# Autodesk Inventor assembly: 1725850 EAGF-V2-KF-100-100---(0)
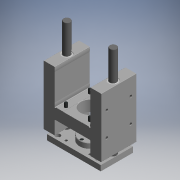
[picture p0: Inventor's stored thumbnail of the model, 180x180]
Saved by Autodesk Inventor 2017.3 (Build 213256000, 256)
## iProperties
Category: PARTsolutions
Company: FESTO
Part Number: 1725850 EAGF-V2-KF-100-100---(0)
Catalog Web Link: www.cadenas.de
Description: EAGF-guide unit
Vendor: FESTO
Document SubType Name: Assembly
Designer: partserver
Manufacturer: FESTO
Mass: 14023 g
Surface Area: 4822.3 cm^2
Volume: 3416.6 cm^3
Density: 4.10438 g/cm^3
Title: 1725850 EAGF-V2-KF-100-100
Author: Cadenas PARTsolutions
Comments: guide unit
PSOL_IDENT_0: {ATYP=ASSISTANT},{DATA=script=$CADENAS_DATA/23d-libs/festo/webfesto.vbb&M_FAMILY=EAGF&M_GROUP=01&M_P
PSOL_IDENT_1: ARTNO=1725850&IDCODE1=EAGF-V2-KF-100-100&IDCODE2=&customer_number_cns=&MATES=1&LOD=HI&LOCKERP=0&SING
PSOL_IDENT_2: LEPART=1}
NB: 1725850 EAGF-V2-KF-100-100---(0)
NN: EAGF
NT: guide unit
NBSYN: $TNR. $TYP.---($HUBST.)
LINA: 1725850 EAGF-V2-KF-100-100
CATALOG: Festo
TNR: 1725850
TYP: EAGF-V2-KF-100-100
HUBST: 0
L1: 362.8
L2: 126.6
L3: 220
L4: 40
L5: 128
L6: 20
L7: 24.5
L8: 89
L9: 0
L10: 15
L11: 39
H1: 213
H2: 200
H3: 89
H4: 150
H5: 131
H6: 172
H7: 150
B1: 130
B2: 120
B3: 89
B4: 89
B5: 89
D1: 87
D2: 25
D3: 18
D4: 11
D5: 70
KK: M20x1.5
G1: M18
G2: M10
G3: M10
T1: 20
T2: 11
SW: 27
CNSMASSEXACT: 14.023
SUPPLIER: FESTO
ARTICLENO: 1725850 EAGF-V2-KF-100-100---(0)
BOMINFO: 1725850 EAGF-V2-KF-100-100
CREATOR: CADENAS GmbH
## Documents named in this file (12)
- e:\temp\worker_18\temp\exporttempdir_1120_80_rasIC\format_0\1725850 EAGF-V2-KF-100-100---(0).iam
- e:\temp\worker_18\temp\exporttempdir_1120_80_rasIC\format_0\2608532 EAGF-V2-KF-100---(F).ipt
- e:\temp\worker_18\temp\exporttempdir_1120_80_rasIC\format_0\247465 FEN-80-SD---(SD).ipt
- e:\temp\worker_18\temp\exporttempdir_1120_80_rasIC\format_0\242770 EAGF 25x35x40---(B).ipt
- e:\temp\worker_18\temp\exporttempdir_1120_80_rasIC\format_0\1558863 EAGF-V2-KF-100---(J).ipt
- e:\temp\worker_18\temp\exporttempdir_1120_80_rasIC\format_0\1559396 EAGF-V2-KF-100---(R).ipt
- e:\temp\worker_18\temp\exporttempdir_1120_80_rasIC\format_0\1559400 EAGF-V2-KF-80_100---(GS).ipt
- e:\temp\worker_18\temp\exporttempdir_1120_80_rasIC\format_0\DIN-913 - M18x20.ipt
- e:\temp\worker_18\temp\exporttempdir_1120_80_rasIC\format_0\2608532 EAGF-100-100-KF---(FST).ipt
- e:\temp\worker_18\temp\exporttempdir_1120_80_rasIC\format_0\DIN-912 - M12x25(F).ipt
- e:\temp\worker_18\temp\exporttempdir_1120_80_rasIC\format_0\DIN-6912 - M12x25(F).ipt
- e:\temp\worker_18\temp\exporttempdir_1120_80_rasIC\format_0\DIN-912 - M10x50(F).ipt
## Components (25 placed, 11 different names)
1. 2608532 EAGF-V2-KF-100---(F):1 — ABSTREIF_V_1_XY@1 <-> ANBAU_XY@2, ABSTREIF_V_1_Z@1 <-> ANBAU_Z@2, ABSTREIF_V_1_YZ@1 <-> ANBAU_YZ@2, ABSTREIF_V_2_XY@1 <-> ANBAU_XY@3, ABSTREIF_V_2_Z@1 <-> ANBAU_Z@3, ABSTREIF_V_2_YZ@1 <-> ANBAU_YZ@3, BUSH_V_1_XY@1 <-> ANBAU_XY@4, BUSH_V_1_Z@1 <-> ANBAU_Z@4, BUSH_V_1_YZ@1 <-> ANBAU_YZ@4, BUSH_V_2_XY@1 <-> ANBAU_XY@5, BUSH_V_2_Z@1 <-> ANBAU_Z@5, BUSH_V_2_YZ@1 <-> ANBAU_YZ@5, ABSTREIF_H_1_XY@1 <-> ANBAU_XY@6, ABSTREIF_H_1_Z@1 <-> ANBAU_Z@6, ABSTREIF_H_1_YZ@1 <-> ANBAU_YZ@6, ABSTREIF_H_2_XY@1 <-> ANBAU_XY@7, ABSTREIF_H_2_Z@1 <-> ANBAU_Z@7, ABSTREIF_H_2_YZ@1 <-> ANBAU_YZ@7, BUSH_H_1_XY@1 <-> ANBAU_XY@8, BUSH_H_1_Z@1 <-> ANBAU_Z@8, BUSH_H_1_YZ@1 <-> ANBAU_YZ@8, BUSH_H_2_XY@1 <-> ANBAU_XY@9, BUSH_H_2_Z@1 <-> ANBAU_Z@9, BUSH_H_2_YZ@1 <-> ANBAU_YZ@9, JOCH_Z@1 <-> ANBAU_Z@10, JOCH_YZ@1 <-> ANBAU_YZ@10, DIN912_1_Z@1 <-> ANBAU_Z@22, DIN912_2_Z@1 <-> ANBAU_Z@23, DIN912_3_Z@1 <-> ANBAU_Z@24, DIN912_4_Z@1 <-> ANBAU_Z@25
2. 247465 FEN-80-SD---(SD):1 — ABSTREIF_V_1_XY@1 <-> ANBAU_XY@2, ABSTREIF_V_1_Z@1 <-> ANBAU_Z@2, ABSTREIF_V_1_YZ@1 <-> ANBAU_YZ@2
3. 247465 FEN-80-SD---(SD):2 — ABSTREIF_V_2_XY@1 <-> ANBAU_XY@3, ABSTREIF_V_2_Z@1 <-> ANBAU_Z@3, ABSTREIF_V_2_YZ@1 <-> ANBAU_YZ@3
4. 242770 EAGF 25x35x40---(B):1 — BUSH_V_1_XY@1 <-> ANBAU_XY@4, BUSH_V_1_Z@1 <-> ANBAU_Z@4, BUSH_V_1_YZ@1 <-> ANBAU_YZ@4
5. 242770 EAGF 25x35x40---(B):2 — BUSH_V_2_XY@1 <-> ANBAU_XY@5, BUSH_V_2_Z@1 <-> ANBAU_Z@5, BUSH_V_2_YZ@1 <-> ANBAU_YZ@5
6. 247465 FEN-80-SD---(SD):3 — ABSTREIF_H_1_XY@1 <-> ANBAU_XY@6, ABSTREIF_H_1_Z@1 <-> ANBAU_Z@6, ABSTREIF_H_1_YZ@1 <-> ANBAU_YZ@6
7. 247465 FEN-80-SD---(SD):4 — ABSTREIF_H_2_XY@1 <-> ANBAU_XY@7, ABSTREIF_H_2_Z@1 <-> ANBAU_Z@7, ABSTREIF_H_2_YZ@1 <-> ANBAU_YZ@7
8. 242770 EAGF 25x35x40---(B):3 — BUSH_H_1_XY@1 <-> ANBAU_XY@8, BUSH_H_1_Z@1 <-> ANBAU_Z@8, BUSH_H_1_YZ@1 <-> ANBAU_YZ@8
9. 242770 EAGF 25x35x40---(B):4 — BUSH_H_2_XY@1 <-> ANBAU_XY@9, BUSH_H_2_Z@1 <-> ANBAU_Z@9, BUSH_H_2_YZ@1 <-> ANBAU_YZ@9
10. 1558863 EAGF-V2-KF-100---(J):1 — JOCH_Z@1 <-> ANBAU_Z@10, JOCH_YZ@1 <-> ANBAU_YZ@10, RING_XY@10 <-> ANBAU_XY@11, RING_Z@10 <-> ANBAU_Z@11, RING_YZ@10 <-> ANBAU_YZ@11, STANGE_XY@10 <-> ANBAU_XY@14, STANGE_Z@10 <-> ANBAU_Z@14, STANGE_2_XY@10 <-> ANBAU_XY@15, STANGE_2_Z@10 <-> ANBAU_Z@15, SCREW_1_XY@10 <-> ANBAU_XY@16, SCREW_1_Z@10 <-> ANBAU_Z@16, SCREW_1_YZ@10 <-> ANBAU_YZ@16, SCREW_2_XY@10 <-> ANBAU_XY@17, SCREW_2_Z@10 <-> ANBAU_Z@17, SCREW_2_YZ@10 <-> ANBAU_YZ@17, SCREW_3_XY@10 <-> ANBAU_XY@18, SCREW_3_Z@10 <-> ANBAU_Z@18, SCREW_3_YZ@10 <-> ANBAU_YZ@18, SCREW_4_XY@10 <-> ANBAU_XY@19, SCREW_4_Z@10 <-> ANBAU_Z@19, SCREW_4_YZ@10 <-> ANBAU_YZ@19, DIN6912_1_XY@10 <-> MONTAGE_XY@20, DIN6912_1_Z@10 <-> MONTAGE_Z@20, DIN6912_2_XY@10 <-> MONTAGE_XY@21, DIN6912_2_Z@10 <-> MONTAGE_Z@21
11. 1559396 EAGF-V2-KF-100---(R):1 — RING_XY@10 <-> ANBAU_XY@11, RING_Z@10 <-> ANBAU_Z@11, RING_YZ@10 <-> ANBAU_YZ@11, EP_IP_XY@11 <-> ANBAU_XY@12, EP_IP_Z@11 <-> ANBAU_Z@12, EP_IP_YZ@11 <-> ANBAU_YZ@12
12. 1559400 EAGF-V2-KF-80_100---(GS):1 — EP_IP_XY@11 <-> ANBAU_XY@12, EP_IP_Z@11 <-> ANBAU_Z@12, EP_IP_YZ@11 <-> ANBAU_YZ@12, EP_IP_Z@12 <-> IP2_Z@13
13. DIN-913 - M18x20:1 — EP_IP_Z@12 <-> IP2_Z@13
14. 2608532 EAGF-100-100-KF---(FST):1 — STANGE_XY@10 <-> ANBAU_XY@14, STANGE_Z@10 <-> ANBAU_Z@14
15. 2608532 EAGF-100-100-KF---(FST):2 — STANGE_2_XY@10 <-> ANBAU_XY@15, STANGE_2_Z@10 <-> ANBAU_Z@15
16. DIN-912 - M12x25(F):1 — SCREW_1_XY@10 <-> ANBAU_XY@16, SCREW_1_Z@10 <-> ANBAU_Z@16, SCREW_1_YZ@10 <-> ANBAU_YZ@16
17. DIN-912 - M12x25(F):2 — SCREW_2_XY@10 <-> ANBAU_XY@17, SCREW_2_Z@10 <-> ANBAU_Z@17, SCREW_2_YZ@10 <-> ANBAU_YZ@17
18. DIN-912 - M12x25(F):3 — SCREW_3_XY@10 <-> ANBAU_XY@18, SCREW_3_Z@10 <-> ANBAU_Z@18, SCREW_3_YZ@10 <-> ANBAU_YZ@18
19. DIN-912 - M12x25(F):4 — SCREW_4_XY@10 <-> ANBAU_XY@19, SCREW_4_Z@10 <-> ANBAU_Z@19, SCREW_4_YZ@10 <-> ANBAU_YZ@19
20. DIN-6912 - M12x25(F):1 — DIN6912_1_XY@10 <-> MONTAGE_XY@20, DIN6912_1_Z@10 <-> MONTAGE_Z@20
21. DIN-6912 - M12x25(F):2 — DIN6912_2_XY@10 <-> MONTAGE_XY@21, DIN6912_2_Z@10 <-> MONTAGE_Z@21
22. DIN-912 - M10x50(F):1 — DIN912_1_Z@1 <-> ANBAU_Z@22
23. DIN-912 - M10x50(F):2 — DIN912_2_Z@1 <-> ANBAU_Z@23
24. DIN-912 - M10x50(F):3 — DIN912_3_Z@1 <-> ANBAU_Z@24
25. DIN-912 - M10x50(F):4 — DIN912_4_Z@1 <-> ANBAU_Z@25
## Relationships (57: Mate 36, Angle 15, Flush 6)
- ABSTREIF_V_1_XY@1 <-> ANBAU_XY@2 [Mate]: 2608532 EAGF-V2-KF-100---(F):1 ↔ 247465 FEN-80-SD---(SD):1
- ABSTREIF_V_1_Z@1 <-> ANBAU_Z@2 [Mate]: 2608532 EAGF-V2-KF-100---(F):1 ↔ 247465 FEN-80-SD---(SD):1
- ABSTREIF_V_1_YZ@1 <-> ANBAU_YZ@2 [Angle] (0 deg): 2608532 EAGF-V2-KF-100---(F):1 ↔ 247465 FEN-80-SD---(SD):1
- ABSTREIF_V_2_XY@1 <-> ANBAU_XY@3 [Mate]: 2608532 EAGF-V2-KF-100---(F):1 ↔ 247465 FEN-80-SD---(SD):2
- ABSTREIF_V_2_Z@1 <-> ANBAU_Z@3 [Mate]: 2608532 EAGF-V2-KF-100---(F):1 ↔ 247465 FEN-80-SD---(SD):2
- ABSTREIF_V_2_YZ@1 <-> ANBAU_YZ@3 [Angle] (0 deg): 2608532 EAGF-V2-KF-100---(F):1 ↔ 247465 FEN-80-SD---(SD):2
- BUSH_V_1_XY@1 <-> ANBAU_XY@4 [Mate]: 2608532 EAGF-V2-KF-100---(F):1 ↔ 242770 EAGF 25x35x40---(B):1
- BUSH_V_1_Z@1 <-> ANBAU_Z@4 [Mate]: 2608532 EAGF-V2-KF-100---(F):1 ↔ 242770 EAGF 25x35x40---(B):1
- BUSH_V_1_YZ@1 <-> ANBAU_YZ@4 [Angle] (0 deg): 2608532 EAGF-V2-KF-100---(F):1 ↔ 242770 EAGF 25x35x40---(B):1
- BUSH_V_2_XY@1 <-> ANBAU_XY@5 [Mate]: 2608532 EAGF-V2-KF-100---(F):1 ↔ 242770 EAGF 25x35x40---(B):2
- BUSH_V_2_Z@1 <-> ANBAU_Z@5 [Mate]: 2608532 EAGF-V2-KF-100---(F):1 ↔ 242770 EAGF 25x35x40---(B):2
- BUSH_V_2_YZ@1 <-> ANBAU_YZ@5 [Angle] (0 deg): 2608532 EAGF-V2-KF-100---(F):1 ↔ 242770 EAGF 25x35x40---(B):2
- ABSTREIF_H_1_XY@1 <-> ANBAU_XY@6 [Mate]: 2608532 EAGF-V2-KF-100---(F):1 ↔ 247465 FEN-80-SD---(SD):3
- ABSTREIF_H_1_Z@1 <-> ANBAU_Z@6 [Mate]: 2608532 EAGF-V2-KF-100---(F):1 ↔ 247465 FEN-80-SD---(SD):3
- ABSTREIF_H_1_YZ@1 <-> ANBAU_YZ@6 [Angle] (0 deg): 2608532 EAGF-V2-KF-100---(F):1 ↔ 247465 FEN-80-SD---(SD):3
- ABSTREIF_H_2_XY@1 <-> ANBAU_XY@7 [Mate]: 2608532 EAGF-V2-KF-100---(F):1 ↔ 247465 FEN-80-SD---(SD):4
- ABSTREIF_H_2_Z@1 <-> ANBAU_Z@7 [Mate]: 2608532 EAGF-V2-KF-100---(F):1 ↔ 247465 FEN-80-SD---(SD):4
- ABSTREIF_H_2_YZ@1 <-> ANBAU_YZ@7 [Angle] (0 deg): 2608532 EAGF-V2-KF-100---(F):1 ↔ 247465 FEN-80-SD---(SD):4
- BUSH_H_1_XY@1 <-> ANBAU_XY@8 [Mate]: 2608532 EAGF-V2-KF-100---(F):1 ↔ 242770 EAGF 25x35x40---(B):3
- BUSH_H_1_Z@1 <-> ANBAU_Z@8 [Mate]: 2608532 EAGF-V2-KF-100---(F):1 ↔ 242770 EAGF 25x35x40---(B):3
- BUSH_H_1_YZ@1 <-> ANBAU_YZ@8 [Angle] (0 deg): 2608532 EAGF-V2-KF-100---(F):1 ↔ 242770 EAGF 25x35x40---(B):3
- BUSH_H_2_XY@1 <-> ANBAU_XY@9 [Mate]: 2608532 EAGF-V2-KF-100---(F):1 ↔ 242770 EAGF 25x35x40---(B):4
- BUSH_H_2_Z@1 <-> ANBAU_Z@9 [Mate]: 2608532 EAGF-V2-KF-100---(F):1 ↔ 242770 EAGF 25x35x40---(B):4
- BUSH_H_2_YZ@1 <-> ANBAU_YZ@9 [Angle] (0 deg): 2608532 EAGF-V2-KF-100---(F):1 ↔ 242770 EAGF 25x35x40---(B):4
- JOCH_Z@1 <-> ANBAU_Z@10 [Mate]: 2608532 EAGF-V2-KF-100---(F):1 ↔ 1558863 EAGF-V2-KF-100---(J):1
- JOCH_YZ@1 <-> ANBAU_YZ@10 [Angle] (0 deg): 2608532 EAGF-V2-KF-100---(F):1 ↔ 1558863 EAGF-V2-KF-100---(J):1
- RING_XY@10 <-> ANBAU_XY@11 [Mate]: 1558863 EAGF-V2-KF-100---(J):1 ↔ 1559396 EAGF-V2-KF-100---(R):1
- RING_Z@10 <-> ANBAU_Z@11 [Mate]: 1558863 EAGF-V2-KF-100---(J):1 ↔ 1559396 EAGF-V2-KF-100---(R):1
- RING_YZ@10 <-> ANBAU_YZ@11 [Angle] (0 deg): 1558863 EAGF-V2-KF-100---(J):1 ↔ 1559396 EAGF-V2-KF-100---(R):1
- EP_IP_XY@11 <-> ANBAU_XY@12 [Mate]: 1559396 EAGF-V2-KF-100---(R):1 ↔ 1559400 EAGF-V2-KF-80_100---(GS):1
- EP_IP_Z@11 <-> ANBAU_Z@12 [Mate]: 1559396 EAGF-V2-KF-100---(R):1 ↔ 1559400 EAGF-V2-KF-80_100---(GS):1
- EP_IP_YZ@11 <-> ANBAU_YZ@12 [Angle] (0 deg): 1559396 EAGF-V2-KF-100---(R):1 ↔ 1559400 EAGF-V2-KF-80_100---(GS):1
- EP_IP_Z@12 <-> IP2_Z@13 [Mate]: 1559400 EAGF-V2-KF-80_100---(GS):1 ↔ DIN-913 - M18x20:1
- STANGE_XY@10 <-> ANBAU_XY@14 [Mate]: 1558863 EAGF-V2-KF-100---(J):1 ↔ 2608532 EAGF-100-100-KF---(FST):1
- STANGE_Z@10 <-> ANBAU_Z@14 [Mate]: 1558863 EAGF-V2-KF-100---(J):1 ↔ 2608532 EAGF-100-100-KF---(FST):1
- STANGE_2_XY@10 <-> ANBAU_XY@15 [Mate]: 1558863 EAGF-V2-KF-100---(J):1 ↔ 2608532 EAGF-100-100-KF---(FST):2
- STANGE_2_Z@10 <-> ANBAU_Z@15 [Mate]: 1558863 EAGF-V2-KF-100---(J):1 ↔ 2608532 EAGF-100-100-KF---(FST):2
- SCREW_1_XY@10 <-> ANBAU_XY@16 [Flush]: 1558863 EAGF-V2-KF-100---(J):1 ↔ DIN-912 - M12x25(F):1
- SCREW_1_Z@10 <-> ANBAU_Z@16 [Mate]: 1558863 EAGF-V2-KF-100---(J):1 ↔ DIN-912 - M12x25(F):1
- SCREW_1_YZ@10 <-> ANBAU_YZ@16 [Angle] (0 deg): 1558863 EAGF-V2-KF-100---(J):1 ↔ DIN-912 - M12x25(F):1
- SCREW_2_XY@10 <-> ANBAU_XY@17 [Flush]: 1558863 EAGF-V2-KF-100---(J):1 ↔ DIN-912 - M12x25(F):2
- SCREW_2_Z@10 <-> ANBAU_Z@17 [Mate]: 1558863 EAGF-V2-KF-100---(J):1 ↔ DIN-912 - M12x25(F):2
- SCREW_2_YZ@10 <-> ANBAU_YZ@17 [Angle] (0 deg): 1558863 EAGF-V2-KF-100---(J):1 ↔ DIN-912 - M12x25(F):2
- SCREW_3_XY@10 <-> ANBAU_XY@18 [Flush]: 1558863 EAGF-V2-KF-100---(J):1 ↔ DIN-912 - M12x25(F):3
- SCREW_3_Z@10 <-> ANBAU_Z@18 [Mate]: 1558863 EAGF-V2-KF-100---(J):1 ↔ DIN-912 - M12x25(F):3
- SCREW_3_YZ@10 <-> ANBAU_YZ@18 [Angle] (0 deg): 1558863 EAGF-V2-KF-100---(J):1 ↔ DIN-912 - M12x25(F):3
- SCREW_4_XY@10 <-> ANBAU_XY@19 [Flush]: 1558863 EAGF-V2-KF-100---(J):1 ↔ DIN-912 - M12x25(F):4
- SCREW_4_Z@10 <-> ANBAU_Z@19 [Mate]: 1558863 EAGF-V2-KF-100---(J):1 ↔ DIN-912 - M12x25(F):4
- SCREW_4_YZ@10 <-> ANBAU_YZ@19 [Angle] (0 deg): 1558863 EAGF-V2-KF-100---(J):1 ↔ DIN-912 - M12x25(F):4
- DIN6912_1_XY@10 <-> MONTAGE_XY@20 [Flush]: 1558863 EAGF-V2-KF-100---(J):1 ↔ DIN-6912 - M12x25(F):1
- DIN6912_1_Z@10 <-> MONTAGE_Z@20 [Mate]: 1558863 EAGF-V2-KF-100---(J):1 ↔ DIN-6912 - M12x25(F):1
- DIN6912_2_XY@10 <-> MONTAGE_XY@21 [Flush]: 1558863 EAGF-V2-KF-100---(J):1 ↔ DIN-6912 - M12x25(F):2
- DIN6912_2_Z@10 <-> MONTAGE_Z@21 [Mate]: 1558863 EAGF-V2-KF-100---(J):1 ↔ DIN-6912 - M12x25(F):2
- DIN912_1_Z@1 <-> ANBAU_Z@22 [Mate]: 2608532 EAGF-V2-KF-100---(F):1 ↔ DIN-912 - M10x50(F):1
- DIN912_2_Z@1 <-> ANBAU_Z@23 [Mate]: 2608532 EAGF-V2-KF-100---(F):1 ↔ DIN-912 - M10x50(F):2
- DIN912_3_Z@1 <-> ANBAU_Z@24 [Mate]: 2608532 EAGF-V2-KF-100---(F):1 ↔ DIN-912 - M10x50(F):3
- DIN912_4_Z@1 <-> ANBAU_Z@25 [Mate]: 2608532 EAGF-V2-KF-100---(F):1 ↔ DIN-912 - M10x50(F):4
